# Autodesk Inventor assembly: populated-keyboard_cherrymx
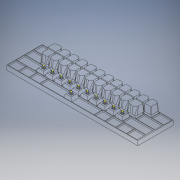
[picture p0: Inventor's stored thumbnail of the model, 180x180]
Saved by Autodesk Inventor 2016 (Build 200138000, 138)
## iProperties
Created: 2016-12-08
Part Number: populated-keyboard_cherrymx
Document SubType Name: Assembly
Designer: Cemra JC
Author: Cemra JC
## Documents named in this file (6)
- J:\The Files\The Software Files\Projects\stenotoppers\cherrymx\base-model\populated-keyboard_cherrymx.iam
- J:\The Files\The Software Files\Projects\stenotoppers\cherrymx\base-model\keyboard-mockup_cherrymx.iam
- J:\The Files\The Software Files\Projects\stenotoppers\cherrymx\base-model\standard-keycap_top-rows_base_cherrymx.ipt
- J:\The Files\The Software Files\Projects\stenotoppers\cherrymx\base-model\keyswitch_cherrymx.iam
- J:\The Files\The Software Files\Projects\stenotoppers\cherrymx\base-model\smaller-keycap_top-rows_base_cherrymx.ipt
- J:\The Files\The Software Files\Projects\stenotoppers\cherrymx\base-model\larger-keycap_top-rows_base_cherrymx.ipt
## Components (25 placed, 5 different names)
1. keyboard-mockup_cherrymx:1 [sub-assembly] — Rigid:3, Rigid:4, Rigid:5, Rigid:6, Rigid:7, Rigid:8, Rigid:9
2. keyswitch_cherrymx:1 [sub-assembly] — Rigid:5
3. smaller-keycap_top-rows_base_cherrymx:1 — Rigid:7
4. smaller-keycap_top-rows_base_cherrymx:2 — Rigid:6
5. larger-keycap_top-rows_base_cherrymx:1 — Rigid:8
6. larger-keycap_top-rows_base_cherrymx:2 — Rigid:9
7. standard-keycap_top-rows_base_cherrymx:4 — Rigid:3
8. standard-keycap_top-rows_base_cherrymx:5
9. standard-keycap_top-rows_base_cherrymx:6
10. standard-keycap_top-rows_base_cherrymx:7
11. standard-keycap_top-rows_base_cherrymx:8
12. standard-keycap_top-rows_base_cherrymx:9
13. standard-keycap_top-rows_base_cherrymx:10
14. standard-keycap_top-rows_base_cherrymx:11
15. standard-keycap_top-rows_base_cherrymx:12
16. standard-keycap_top-rows_base_cherrymx:13
17. standard-keycap_top-rows_base_cherrymx:2 — Rigid:4
18. standard-keycap_top-rows_base_cherrymx:14
19. standard-keycap_top-rows_base_cherrymx:15
20. standard-keycap_top-rows_base_cherrymx:16
21. standard-keycap_top-rows_base_cherrymx:17
22. standard-keycap_top-rows_base_cherrymx:18
23. standard-keycap_top-rows_base_cherrymx:19
24. standard-keycap_top-rows_base_cherrymx:20
25. standard-keycap_top-rows_base_cherrymx:21
## Component patterns: (10 elements, first: standard-keycap_top-rows_base_cherrymx:4), (9 elements, first: standard-keycap_top-rows_base_cherrymx:2)
## Relationships (7: WeldJoint 7)
- Rigid:3 [WeldJoint]: keyboard-mockup_cherrymx:1 ↔ standard-keycap_top-rows_base_cherrymx:4
- Rigid:4 [WeldJoint]: keyboard-mockup_cherrymx:1 ↔ standard-keycap_top-rows_base_cherrymx:2
- Rigid:5 [WeldJoint]: keyboard-mockup_cherrymx:1 ↔ keyswitch_cherrymx:1
- Rigid:6 [WeldJoint]: keyboard-mockup_cherrymx:1 ↔ smaller-keycap_top-rows_base_cherrymx:2
- Rigid:7 [WeldJoint]: keyboard-mockup_cherrymx:1 ↔ smaller-keycap_top-rows_base_cherrymx:1
- Rigid:8 [WeldJoint]: keyboard-mockup_cherrymx:1 ↔ larger-keycap_top-rows_base_cherrymx:1
- Rigid:9 [WeldJoint]: keyboard-mockup_cherrymx:1 ↔ larger-keycap_top-rows_base_cherrymx:2
